# Autodesk Inventor assembly: LegAssembly_MIR
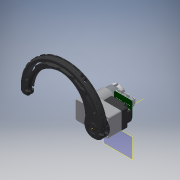
[picture p0: Inventor's stored thumbnail of the model, 180x180]
Saved by Autodesk Inventor 2016 (Build 200138000, 138)
## iProperties
Created: 2016-11-06
Part Number: LegAssembly_MIR
Document SubType Name: Assembly
Designer: brent
Author: brent
## Documents named in this file (7)
- C:\Users\brent\OneDrive\classes\desinv22\final\leggedbot_mechanical\LegAssembly_MIR.iam
- C:\Users\brent\OneDrive\classes\desinv22\final\leggedbot_mechanical\offtheshelf\AS5048B_Breakout_MIR.ipt
- C:\Users\brent\OneDrive\classes\desinv22\final\leggedbot_mechanical\offtheshelf\Pololu_120to1Offset_MIR.ipt
- C:\Users\brent\OneDrive\classes\desinv22\final\leggedbot_mechanical\offtheshelf\DiametricMagnet_625_MIR.ipt
- C:\Users\brent\OneDrive\classes\desinv22\final\leggedbot_mechanical\MagnetHolder_MIR.ipt
- C:\Users\brent\OneDrive\classes\desinv22\final\leggedbot_mechanical\EncoderMount_MIR.ipt
- C:\Users\brent\OneDrive\classes\desinv22\final\leggedbot_mechanical\Leg_MIR.ipt
## Components (6 placed, 6 different names)
1. AS5048B_Breakout_MIR:1 — Mate:3, Mate:2, Angle:1
2. Pololu_120to1Offset_MIR:1 — Flush:5, Mate:3, Mate:2, Flush:1, Angle:1, Mate:5, Mate:4, Flush:2, Flush:4, Flush:3, Mate:7, Mate:6
3. DiametricMagnet_625_MIR:1 — Mate:5, Mate:4
4. MagnetHolder_MIR:1 — Flush:2
5. EncoderMount_MIR:1 — Flush:4, Flush:3
6. Leg_MIR:1 — Mate:7, Mate:6
## Relationships (12: Mate 10, Flush 1, Angle 1)
- Flush:5: Pololu_120to1Offset_MIR:1
- Mate:3 (-3.5 mm): AS5048B_Breakout_MIR:1 ↔ Pololu_120to1Offset_MIR:1
- Mate:2: AS5048B_Breakout_MIR:1 ↔ Pololu_120to1Offset_MIR:1
- Flush:1 [Mate]: Pololu_120to1Offset_MIR:1
- Angle:1 (0 deg): AS5048B_Breakout_MIR:1 ↔ Pololu_120to1Offset_MIR:1
- Mate:5: Pololu_120to1Offset_MIR:1 ↔ DiametricMagnet_625_MIR:1
- Mate:4: Pololu_120to1Offset_MIR:1 ↔ DiametricMagnet_625_MIR:1
- Flush:2 [Mate]: Pololu_120to1Offset_MIR:1 ↔ MagnetHolder_MIR:1
- Flush:4 [Mate]: Pololu_120to1Offset_MIR:1 ↔ EncoderMount_MIR:1
- Flush:3 [Mate]: Pololu_120to1Offset_MIR:1 ↔ EncoderMount_MIR:1
- Mate:7: Pololu_120to1Offset_MIR:1 ↔ Leg_MIR:1
- Mate:6 (0.2 mm): Pololu_120to1Offset_MIR:1 ↔ Leg_MIR:1
